# Autodesk Inventor assembly: BasicFramework
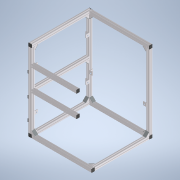
[picture p0: Inventor's stored thumbnail of the model, 180x180]
Saved by Autodesk Inventor 2020 (Build 240168000, 168)
## iProperties
Created: 2019-11-06
Part Number: BasicFramework
Document SubType Name: Assembly
Designer: nicoc
Author: nicoc
## Documents named in this file (10)
- D:\03_Bachelor\Semester_5\pro5E\Stand\CAD\Version2\BasicFramework\BasicFramework.iam
- D:\03_Bachelor\Semester_5\pro5E\Stand\CAD\Version2\BasicFramework\item_7000009_Profile_8_40x40_E_L=736_3.ipt
- D:\03_Bachelor\Semester_5\pro5E\Stand\CAD\Version2\BasicFramework\item_7000009_Profile_8_40x40_E_L=742_2.ipt
- D:\03_Bachelor\Semester_5\pro5E\Stand\CAD\Version2\BasicFramework\item_0002601_Cap_8_40x40_2.ipt
- D:\03_Bachelor\Semester_5\pro5E\Stand\CAD\Version2\BasicFramework\item_7000009_Profile_8_40x40_E_L=920_1.ipt
- D:\03_Bachelor\Semester_5\pro5E\Stand\CAD\Version2\BasicFramework\item_7000009_Profile_8_40x40_E_L=670_1.ipt
- D:\03_Bachelor\Semester_5\pro5E\Stand\CAD\Version2\BasicFramework\item_7000009_Profile_8_40x40_E_L=550_2.ipt
- D:\03_Bachelor\Semester_5\pro5E\Stand\CAD\Version2\BasicFramework\AngleBracket40x40\item_0067011_Angle_Bracket_Set_8_40x40_4.iam
- D:\03_Bachelor\Semester_5\pro5E\Stand\CAD\Version2\BasicFramework\BracketPanel\item_0048628_Angle_Bracket_V_8_40_Zn_1.iam
- D:\03_Bachelor\Semester_5\pro5E\Stand\CAD\Version2\BasicFramework\UniversalHolder\item_0062790_Universal_Holder_with_Securing_Strap_8_180_1.iam
## Components (43 placed, 9 different names)
1. item_7000009_Profile_8_40x40_E_L=736_3:1 — Mate:1, Flush:1, Flush:2, Mate:5, Flush:9, Flush:10, Mate:13, Mate:52, Mate:54, Flush:62
2. item_7000009_Profile_8_40x40_E_L=742_2:2 — Mate:3, Flush:5, Flush:6, Mate:4, Flush:7, Flush:8, Mate:5, Flush:9, Mate:6, Flush:12, Mate:10, Flush:19, Mate:39, Mate:42, Flush:56
3. item_0002601_Cap_8_40x40_2:2 — Mate:1, Flush:1, Flush:2
4. item_0002601_Cap_8_40x40_2:4 — Mate:3, Flush:5, Flush:6, Flush:10, Flush:11
5. item_0002601_Cap_8_40x40_2:5 — Mate:4, Flush:7, Flush:8, Flush:20
6. item_7000009_Profile_8_40x40_E_L=920_1:1 — Mate:6, Flush:11, Flush:12, Mate:9, Flush:17, Flush:18, Mate:21, Mate:40, Flush:55, Mate:43, Mate:55, Mate:56, Mate:81, Flush:85, Mate:84, Flush:88, Mate:85, Flush:90, Mate:87, Flush:94
7. item_7000009_Profile_8_40x40_E_L=742_2:3 — Mate:9, Flush:17, Mate:12, Flush:24, Flush:29, Mate:15, Flush:42, Mate:37, Mate:41, Flush:76, Flush:79, Flush:91, Flush:93, Flush:95, Flush:97
8. item_0002601_Cap_8_40x40_2:6 — Flush:18, Flush:23
9. item_0002601_Cap_8_40x40_2:7 — Flush:30
10. item_7000009_Profile_8_40x40_E_L=920_1:2 — Mate:10, Flush:19, Flush:20, Flush:33, Mate:17, Flush:39, Mate:20, Flush:41, Mate:36, Flush:53, Mate:38, Flush:54, Mate:70, Flush:77, Mate:71, Flush:78, Mate:72, Flush:80, Mate:77, Mate:80, Mate:86, Flush:92, Mate:88, Flush:96
11. item_7000009_Profile_8_40x40_E_L=736_3:2 — Mate:12, Flush:23, Flush:24, Flush:26, Mate:16, Mate:57, Flush:63, Mate:59, Flush:87, Flush:89
12. item_0002601_Cap_8_40x40_2:8 — Flush:25
13. item_7000009_Profile_8_40x40_E_L=920_1:3 — Flush:25, Flush:26, Mate:13, Mate:53, Flush:61, Mate:58, Flush:64, Mate:74, Flush:81, Mate:83, Flush:86
14. item_7000009_Profile_8_40x40_E_L=736_3:3 — Flush:29, Flush:30, Mate:15, Flush:31, Flush:34, Flush:40, Mate:76, Flush:82, Mate:78, Flush:83
15. item_0002601_Cap_8_40x40_2:9 — Flush:32
16. item_7000009_Profile_8_40x40_E_L=670_1:1 — Flush:31, Flush:32, Mate:16, Mate:73, Mate:75
17. item_7000009_Profile_8_40x40_E_L=550_2:1 — Flush:33, Mate:17, Flush:34, Flush:35, Mate:18, Flush:36
18. item_0002601_Cap_8_40x40_2:10 — Flush:35, Mate:18, Flush:36
19. item_7000009_Profile_8_40x40_E_L=550_2:2 — Flush:39, Mate:20, Flush:40
20. item_0002601_Cap_8_40x40_2:11
21. item_7000009_Profile_8_40x40_E_L=670_1:2 — Flush:41, Mate:21, Flush:42, Mate:79, Flush:84, Mate:82
22. item_0067011_Angle_Bracket_Set_8_40x40_4:1 [sub-assembly] — Mate:36, Mate:37, Flush:53
23. item_0067011_Angle_Bracket_Set_8_40x40_4:2 [sub-assembly] — Mate:38, Mate:39, Flush:54
24. item_0067011_Angle_Bracket_Set_8_40x40_4:5 [sub-assembly] — Mate:42, Mate:43, Flush:56
25. item_0067011_Angle_Bracket_Set_8_40x40_4:8 [sub-assembly] — Mate:40, Mate:41, Flush:55
26. item_0067011_Angle_Bracket_Set_8_40x40_4:9 [sub-assembly] — Mate:52, Mate:53, Flush:61
27. item_0067011_Angle_Bracket_Set_8_40x40_4:10 [sub-assembly] — Mate:54, Mate:55, Flush:62
28. item_0067011_Angle_Bracket_Set_8_40x40_4:11 [sub-assembly] — Mate:56, Mate:57, Flush:63
29. item_0067011_Angle_Bracket_Set_8_40x40_4:12 [sub-assembly] — Mate:58, Mate:59, Flush:64
30. item_0062790_Universal_Holder_with_Securing_Strap_8_180_1:1 [sub-assembly] — Mate:70, Flush:76, Flush:77
31. item_0062790_Universal_Holder_with_Securing_Strap_8_180_1:2 [sub-assembly] — Mate:71, Flush:78, Flush:79
32. item_0062790_Universal_Holder_with_Securing_Strap_8_180_1:3 [sub-assembly] — Mate:72, Flush:80
33. item_0067011_Angle_Bracket_Set_8_40x40_4:13 [sub-assembly] — Mate:73, Mate:74, Flush:81
34. item_0067011_Angle_Bracket_Set_8_40x40_4:14 [sub-assembly] — Mate:75, Mate:76, Flush:82
35. item_0067011_Angle_Bracket_Set_8_40x40_4:15 [sub-assembly] — Mate:77, Mate:78, Flush:83
36. item_0067011_Angle_Bracket_Set_8_40x40_4:16 [sub-assembly] — Mate:79, Mate:80, Flush:84
37. item_0067011_Angle_Bracket_Set_8_40x40_4:17 [sub-assembly] — Mate:81, Mate:82, Flush:85
38. item_0048628_Angle_Bracket_V_8_40_Zn_1:1 [sub-assembly] — Mate:83, Flush:86, Flush:87
39. item_0048628_Angle_Bracket_V_8_40_Zn_1:2 [sub-assembly] — Mate:84, Flush:88, Flush:89
40. item_0048628_Angle_Bracket_V_8_40_Zn_1:3 [sub-assembly] — Mate:85, Flush:90, Flush:91
41. item_0048628_Angle_Bracket_V_8_40_Zn_1:4 [sub-assembly] — Mate:86, Flush:92, Flush:93
42. item_0048628_Angle_Bracket_V_8_40_Zn_1:5 [sub-assembly] — Mate:87, Flush:94, Flush:95
43. item_0048628_Angle_Bracket_V_8_40_Zn_1:6 [sub-assembly] — Mate:88, Flush:96, Flush:97
## Relationships (125: Flush 70, Mate 55)
- Mate:1: item_7000009_Profile_8_40x40_E_L=736_3:1 ↔ item_0002601_Cap_8_40x40_2:2
- Flush:1: item_7000009_Profile_8_40x40_E_L=736_3:1 ↔ item_0002601_Cap_8_40x40_2:2
- Flush:2: item_7000009_Profile_8_40x40_E_L=736_3:1 ↔ item_0002601_Cap_8_40x40_2:2
- Mate:3: item_7000009_Profile_8_40x40_E_L=742_2:2 ↔ item_0002601_Cap_8_40x40_2:4
- Flush:5: item_7000009_Profile_8_40x40_E_L=742_2:2 ↔ item_0002601_Cap_8_40x40_2:4
- Flush:6: item_7000009_Profile_8_40x40_E_L=742_2:2 ↔ item_0002601_Cap_8_40x40_2:4
- Mate:4: item_7000009_Profile_8_40x40_E_L=742_2:2 ↔ item_0002601_Cap_8_40x40_2:5
- Flush:7: item_7000009_Profile_8_40x40_E_L=742_2:2 ↔ item_0002601_Cap_8_40x40_2:5
- Flush:8: item_7000009_Profile_8_40x40_E_L=742_2:2 ↔ item_0002601_Cap_8_40x40_2:5
- Mate:5: item_7000009_Profile_8_40x40_E_L=736_3:1 ↔ item_7000009_Profile_8_40x40_E_L=742_2:2
- Flush:9: item_7000009_Profile_8_40x40_E_L=736_3:1 ↔ item_7000009_Profile_8_40x40_E_L=742_2:2
- Flush:10: item_7000009_Profile_8_40x40_E_L=736_3:1 ↔ item_0002601_Cap_8_40x40_2:4
- Mate:6: item_7000009_Profile_8_40x40_E_L=742_2:2 ↔ item_7000009_Profile_8_40x40_E_L=920_1:1
- Flush:11: item_0002601_Cap_8_40x40_2:4 ↔ item_7000009_Profile_8_40x40_E_L=920_1:1
- Flush:12: item_7000009_Profile_8_40x40_E_L=742_2:2 ↔ item_7000009_Profile_8_40x40_E_L=920_1:1
- [Mate]: item_7000009_Profile_8_40x40_E_L=742_2:3 ↔ item_0002601_Cap_8_40x40_2:6
- [Flush]: item_7000009_Profile_8_40x40_E_L=742_2:3 ↔ item_0002601_Cap_8_40x40_2:6
- [Flush]: item_7000009_Profile_8_40x40_E_L=742_2:3 ↔ item_0002601_Cap_8_40x40_2:6
- [Mate]: item_7000009_Profile_8_40x40_E_L=742_2:3 ↔ item_0002601_Cap_8_40x40_2:7
- [Flush]: item_7000009_Profile_8_40x40_E_L=742_2:3 ↔ item_0002601_Cap_8_40x40_2:7
- [Flush]: item_7000009_Profile_8_40x40_E_L=742_2:3 ↔ item_0002601_Cap_8_40x40_2:7
- Mate:9: item_7000009_Profile_8_40x40_E_L=920_1:1 ↔ item_7000009_Profile_8_40x40_E_L=742_2:3
- Flush:17: item_7000009_Profile_8_40x40_E_L=920_1:1 ↔ item_7000009_Profile_8_40x40_E_L=742_2:3
- Flush:18: item_7000009_Profile_8_40x40_E_L=920_1:1 ↔ item_0002601_Cap_8_40x40_2:6
- Mate:10: item_7000009_Profile_8_40x40_E_L=742_2:2 ↔ item_7000009_Profile_8_40x40_E_L=920_1:2
- Flush:19: item_7000009_Profile_8_40x40_E_L=742_2:2 ↔ item_7000009_Profile_8_40x40_E_L=920_1:2
- Flush:20: item_0002601_Cap_8_40x40_2:5 ↔ item_7000009_Profile_8_40x40_E_L=920_1:2
- [Mate]: item_7000009_Profile_8_40x40_E_L=736_3:2 ↔ item_0002601_Cap_8_40x40_2:8
- [Flush]: item_7000009_Profile_8_40x40_E_L=736_3:2 ↔ item_0002601_Cap_8_40x40_2:8
- [Flush]: item_7000009_Profile_8_40x40_E_L=736_3:2 ↔ item_0002601_Cap_8_40x40_2:8
- Mate:12: item_7000009_Profile_8_40x40_E_L=742_2:3 ↔ item_7000009_Profile_8_40x40_E_L=736_3:2
- Flush:23: item_0002601_Cap_8_40x40_2:6 ↔ item_7000009_Profile_8_40x40_E_L=736_3:2
- Flush:24: item_7000009_Profile_8_40x40_E_L=742_2:3 ↔ item_7000009_Profile_8_40x40_E_L=736_3:2
- Flush:25: item_0002601_Cap_8_40x40_2:8 ↔ item_7000009_Profile_8_40x40_E_L=920_1:3
- Flush:26: item_7000009_Profile_8_40x40_E_L=736_3:2 ↔ item_7000009_Profile_8_40x40_E_L=920_1:3
- Mate:13: item_7000009_Profile_8_40x40_E_L=736_3:1 ↔ item_7000009_Profile_8_40x40_E_L=920_1:3
- [Mate]: item_7000009_Profile_8_40x40_E_L=736_3:3 ↔ item_0002601_Cap_8_40x40_2:9
- [Flush]: item_7000009_Profile_8_40x40_E_L=736_3:3 ↔ item_0002601_Cap_8_40x40_2:9
- [Flush]: item_7000009_Profile_8_40x40_E_L=736_3:3 ↔ item_0002601_Cap_8_40x40_2:9
- Flush:29: item_7000009_Profile_8_40x40_E_L=742_2:3 ↔ item_7000009_Profile_8_40x40_E_L=736_3:3
- Flush:30: item_0002601_Cap_8_40x40_2:7 ↔ item_7000009_Profile_8_40x40_E_L=736_3:3
- Mate:15: item_7000009_Profile_8_40x40_E_L=742_2:3 ↔ item_7000009_Profile_8_40x40_E_L=736_3:3
- Flush:31: item_7000009_Profile_8_40x40_E_L=736_3:3 ↔ item_7000009_Profile_8_40x40_E_L=670_1:1
- Flush:32: item_0002601_Cap_8_40x40_2:9 ↔ item_7000009_Profile_8_40x40_E_L=670_1:1
- Mate:16: item_7000009_Profile_8_40x40_E_L=736_3:2 ↔ item_7000009_Profile_8_40x40_E_L=670_1:1
- Flush:33: item_7000009_Profile_8_40x40_E_L=920_1:2 ↔ item_7000009_Profile_8_40x40_E_L=550_2:1
- Mate:17: item_7000009_Profile_8_40x40_E_L=920_1:2 ↔ item_7000009_Profile_8_40x40_E_L=550_2:1
- Flush:34 (480 mm): item_7000009_Profile_8_40x40_E_L=736_3:3 ↔ item_7000009_Profile_8_40x40_E_L=550_2:1
- Flush:35: item_7000009_Profile_8_40x40_E_L=550_2:1 ↔ item_0002601_Cap_8_40x40_2:10
- Mate:18: item_7000009_Profile_8_40x40_E_L=550_2:1 ↔ item_0002601_Cap_8_40x40_2:10
- Flush:36: item_7000009_Profile_8_40x40_E_L=550_2:1 ↔ item_0002601_Cap_8_40x40_2:10
- [Flush]: item_7000009_Profile_8_40x40_E_L=550_2:2 ↔ item_0002601_Cap_8_40x40_2:11
- [Mate]: item_7000009_Profile_8_40x40_E_L=550_2:2 ↔ item_0002601_Cap_8_40x40_2:11
- [Flush]: item_7000009_Profile_8_40x40_E_L=550_2:2 ↔ item_0002601_Cap_8_40x40_2:11
- Flush:39: item_7000009_Profile_8_40x40_E_L=920_1:2 ↔ item_7000009_Profile_8_40x40_E_L=550_2:2
- Mate:20: item_7000009_Profile_8_40x40_E_L=920_1:2 ↔ item_7000009_Profile_8_40x40_E_L=550_2:2
- Flush:40 (750 mm): item_7000009_Profile_8_40x40_E_L=736_3:3 ↔ item_7000009_Profile_8_40x40_E_L=550_2:2
- Flush:41: item_7000009_Profile_8_40x40_E_L=920_1:2 ↔ item_7000009_Profile_8_40x40_E_L=670_1:2
- Mate:21: item_7000009_Profile_8_40x40_E_L=920_1:1 ↔ item_7000009_Profile_8_40x40_E_L=670_1:2
- Flush:42 (480 mm): item_7000009_Profile_8_40x40_E_L=742_2:3 ↔ item_7000009_Profile_8_40x40_E_L=670_1:2
- Mate:36: item_7000009_Profile_8_40x40_E_L=920_1:2 ↔ item_0067011_Angle_Bracket_Set_8_40x40_4:1
- Mate:37: item_7000009_Profile_8_40x40_E_L=742_2:3 ↔ item_0067011_Angle_Bracket_Set_8_40x40_4:1
- Flush:53: item_7000009_Profile_8_40x40_E_L=920_1:2 ↔ item_0067011_Angle_Bracket_Set_8_40x40_4:1
- Mate:38: item_7000009_Profile_8_40x40_E_L=920_1:2 ↔ item_0067011_Angle_Bracket_Set_8_40x40_4:2
- Mate:39: item_7000009_Profile_8_40x40_E_L=742_2:2 ↔ item_0067011_Angle_Bracket_Set_8_40x40_4:2
- Flush:54: item_7000009_Profile_8_40x40_E_L=920_1:2 ↔ item_0067011_Angle_Bracket_Set_8_40x40_4:2
- Mate:40: item_7000009_Profile_8_40x40_E_L=920_1:1 ↔ item_0067011_Angle_Bracket_Set_8_40x40_4:8
- Mate:41: item_7000009_Profile_8_40x40_E_L=742_2:3 ↔ item_0067011_Angle_Bracket_Set_8_40x40_4:8
- Flush:55: item_7000009_Profile_8_40x40_E_L=920_1:1 ↔ item_0067011_Angle_Bracket_Set_8_40x40_4:8
- Mate:42: item_7000009_Profile_8_40x40_E_L=742_2:2 ↔ item_0067011_Angle_Bracket_Set_8_40x40_4:5
- Mate:43: item_7000009_Profile_8_40x40_E_L=920_1:1 ↔ item_0067011_Angle_Bracket_Set_8_40x40_4:5
- Flush:56: item_7000009_Profile_8_40x40_E_L=742_2:2 ↔ item_0067011_Angle_Bracket_Set_8_40x40_4:5
- Mate:52: item_7000009_Profile_8_40x40_E_L=736_3:1 ↔ item_0067011_Angle_Bracket_Set_8_40x40_4:9
- Mate:53: item_7000009_Profile_8_40x40_E_L=920_1:3 ↔ item_0067011_Angle_Bracket_Set_8_40x40_4:9
- Flush:61: item_7000009_Profile_8_40x40_E_L=920_1:3 ↔ item_0067011_Angle_Bracket_Set_8_40x40_4:9
- Mate:54: item_7000009_Profile_8_40x40_E_L=736_3:1 ↔ item_0067011_Angle_Bracket_Set_8_40x40_4:10
- Mate:55: item_7000009_Profile_8_40x40_E_L=920_1:1 ↔ item_0067011_Angle_Bracket_Set_8_40x40_4:10
- Flush:62: item_7000009_Profile_8_40x40_E_L=736_3:1 ↔ item_0067011_Angle_Bracket_Set_8_40x40_4:10
- Mate:56: item_7000009_Profile_8_40x40_E_L=920_1:1 ↔ item_0067011_Angle_Bracket_Set_8_40x40_4:11
- Mate:57: item_7000009_Profile_8_40x40_E_L=736_3:2 ↔ item_0067011_Angle_Bracket_Set_8_40x40_4:11
- Flush:63: item_7000009_Profile_8_40x40_E_L=736_3:2 ↔ item_0067011_Angle_Bracket_Set_8_40x40_4:11
- Mate:58: item_7000009_Profile_8_40x40_E_L=920_1:3 ↔ item_0067011_Angle_Bracket_Set_8_40x40_4:12
- Mate:59: item_7000009_Profile_8_40x40_E_L=736_3:2 ↔ item_0067011_Angle_Bracket_Set_8_40x40_4:12
- Flush:64: item_7000009_Profile_8_40x40_E_L=920_1:3 ↔ item_0067011_Angle_Bracket_Set_8_40x40_4:12
- Mate:70: item_7000009_Profile_8_40x40_E_L=920_1:2 ↔ item_0062790_Universal_Holder_with_Securing_Strap_8_180_1:1
- Flush:76 (150 mm): item_7000009_Profile_8_40x40_E_L=742_2:3 ↔ item_0062790_Universal_Holder_with_Securing_Strap_8_180_1:1
- Flush:77 (10 mm): item_7000009_Profile_8_40x40_E_L=920_1:2 ↔ item_0062790_Universal_Holder_with_Securing_Strap_8_180_1:1
- Mate:71: item_7000009_Profile_8_40x40_E_L=920_1:2 ↔ item_0062790_Universal_Holder_with_Securing_Strap_8_180_1:2
- Flush:78 (10 mm): item_7000009_Profile_8_40x40_E_L=920_1:2 ↔ item_0062790_Universal_Holder_with_Securing_Strap_8_180_1:2
- Flush:79 (400 mm): item_7000009_Profile_8_40x40_E_L=742_2:3 ↔ item_0062790_Universal_Holder_with_Securing_Strap_8_180_1:2
- Mate:72: item_7000009_Profile_8_40x40_E_L=920_1:2 ↔ item_0062790_Universal_Holder_with_Securing_Strap_8_180_1:3
- Flush:80 (10 mm): item_7000009_Profile_8_40x40_E_L=920_1:2 ↔ item_0062790_Universal_Holder_with_Securing_Strap_8_180_1:3
- Mate:73: item_7000009_Profile_8_40x40_E_L=670_1:1 ↔ item_0067011_Angle_Bracket_Set_8_40x40_4:13
- Mate:74: item_7000009_Profile_8_40x40_E_L=920_1:3 ↔ item_0067011_Angle_Bracket_Set_8_40x40_4:13
- Flush:81: item_7000009_Profile_8_40x40_E_L=920_1:3 ↔ item_0067011_Angle_Bracket_Set_8_40x40_4:13
- Mate:75: item_7000009_Profile_8_40x40_E_L=670_1:1 ↔ item_0067011_Angle_Bracket_Set_8_40x40_4:14
- Mate:76: item_7000009_Profile_8_40x40_E_L=736_3:3 ↔ item_0067011_Angle_Bracket_Set_8_40x40_4:14
- Flush:82: item_7000009_Profile_8_40x40_E_L=736_3:3 ↔ item_0067011_Angle_Bracket_Set_8_40x40_4:14
- Mate:77: item_7000009_Profile_8_40x40_E_L=920_1:2 ↔ item_0067011_Angle_Bracket_Set_8_40x40_4:15
- Mate:78: item_7000009_Profile_8_40x40_E_L=736_3:3 ↔ item_0067011_Angle_Bracket_Set_8_40x40_4:15
- Flush:83: item_7000009_Profile_8_40x40_E_L=736_3:3 ↔ item_0067011_Angle_Bracket_Set_8_40x40_4:15
- Mate:79: item_7000009_Profile_8_40x40_E_L=670_1:2 ↔ item_0067011_Angle_Bracket_Set_8_40x40_4:16
- Mate:80: item_7000009_Profile_8_40x40_E_L=920_1:2 ↔ item_0067011_Angle_Bracket_Set_8_40x40_4:16
- Flush:84: item_7000009_Profile_8_40x40_E_L=670_1:2 ↔ item_0067011_Angle_Bracket_Set_8_40x40_4:16
- Mate:81: item_7000009_Profile_8_40x40_E_L=920_1:1 ↔ item_0067011_Angle_Bracket_Set_8_40x40_4:17
- Mate:82: item_7000009_Profile_8_40x40_E_L=670_1:2 ↔ item_0067011_Angle_Bracket_Set_8_40x40_4:17
- Flush:85: item_7000009_Profile_8_40x40_E_L=920_1:1 ↔ item_0067011_Angle_Bracket_Set_8_40x40_4:17
- Mate:83: item_7000009_Profile_8_40x40_E_L=920_1:3 ↔ item_0048628_Angle_Bracket_V_8_40_Zn_1:1
- Flush:86: item_7000009_Profile_8_40x40_E_L=920_1:3 ↔ item_0048628_Angle_Bracket_V_8_40_Zn_1:1
- Flush:87 (330 mm): item_7000009_Profile_8_40x40_E_L=736_3:2 ↔ item_0048628_Angle_Bracket_V_8_40_Zn_1:1
- Mate:84: item_7000009_Profile_8_40x40_E_L=920_1:1 ↔ item_0048628_Angle_Bracket_V_8_40_Zn_1:2
- Flush:88: item_7000009_Profile_8_40x40_E_L=920_1:1 ↔ item_0048628_Angle_Bracket_V_8_40_Zn_1:2
- Flush:89 (330 mm): item_7000009_Profile_8_40x40_E_L=736_3:2 ↔ item_0048628_Angle_Bracket_V_8_40_Zn_1:2
- Mate:85: item_7000009_Profile_8_40x40_E_L=920_1:1 ↔ item_0048628_Angle_Bracket_V_8_40_Zn_1:3
- Flush:90: item_7000009_Profile_8_40x40_E_L=920_1:1 ↔ item_0048628_Angle_Bracket_V_8_40_Zn_1:3
- Flush:91 (230 mm): item_7000009_Profile_8_40x40_E_L=742_2:3 ↔ item_0048628_Angle_Bracket_V_8_40_Zn_1:3
- Mate:86: item_7000009_Profile_8_40x40_E_L=920_1:2 ↔ item_0048628_Angle_Bracket_V_8_40_Zn_1:4
- Flush:92: item_7000009_Profile_8_40x40_E_L=920_1:2 ↔ item_0048628_Angle_Bracket_V_8_40_Zn_1:4
- Flush:93 (230 mm): item_7000009_Profile_8_40x40_E_L=742_2:3 ↔ item_0048628_Angle_Bracket_V_8_40_Zn_1:4
- Mate:87: item_7000009_Profile_8_40x40_E_L=920_1:1 ↔ item_0048628_Angle_Bracket_V_8_40_Zn_1:5
- Flush:94: item_7000009_Profile_8_40x40_E_L=920_1:1 ↔ item_0048628_Angle_Bracket_V_8_40_Zn_1:5
- Flush:95 (730 mm): item_7000009_Profile_8_40x40_E_L=742_2:3 ↔ item_0048628_Angle_Bracket_V_8_40_Zn_1:5
- Mate:88: item_7000009_Profile_8_40x40_E_L=920_1:2 ↔ item_0048628_Angle_Bracket_V_8_40_Zn_1:6
- Flush:96: item_7000009_Profile_8_40x40_E_L=920_1:2 ↔ item_0048628_Angle_Bracket_V_8_40_Zn_1:6
- Flush:97 (730 mm): item_7000009_Profile_8_40x40_E_L=742_2:3 ↔ item_0048628_Angle_Bracket_V_8_40_Zn_1:6
## Named parameters: d18_d6 = 0 mm, d19_d7 = 0 mm, d20_d8 = 0 mm, d21_d9 = 0 mm, d22_d10 = 0 mm, d23_d11 = 0 mm, d30_d0 = 0 mm, d31_d1 = 0 mm, d32_d2 = 0 mm, d39_d30_d0 = 0 mm, d40_d31_d1 = 0 mm, d41_d32_d2 = 0 mm, d54_d51 = 0 mm, d55_d52 = 0 mm, d56_d53 = 0 mm
